# Autodesk Inventor assembly: Additional_Building
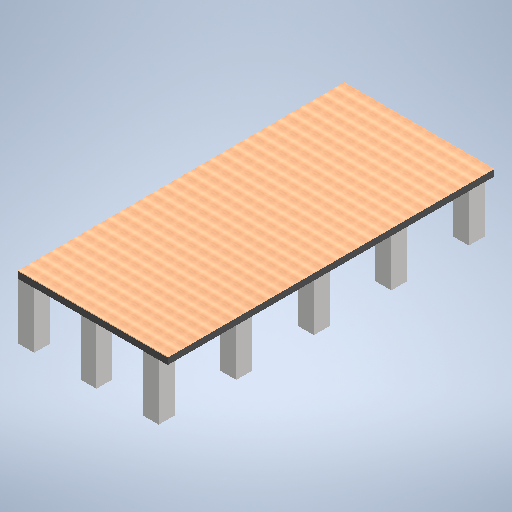
[picture p0: Inventor's stored thumbnail of the model, 512x512]
Saved by Autodesk Inventor 2025 (Build 290162010, 162A)
## iProperties
Created: 2024-08-02
Part Number: Additional_Building
Document SubType Name: Assembly
Designer: Tom
Author: Tom
## Documents named in this file (3)
- C:\Users\Tom\Documents\Inventor\Mobility\Additional_Building\Additional_Building.iam
- C:\Users\Tom\Documents\Inventor\Mobility\Additional_Building\Grid_Of_Piers.iam
- C:\Users\Tom\Documents\Inventor\Mobility\Additional_Building\Floor_System.iam
## Components (2 placed, 2 different names)
1. Grid_Of_Piers:1 [sub-assembly] — Mate:12, Mate:13, Flush:7
2. Floor_System:1 [sub-assembly] — Mate:12, Mate:13, Flush:7
## Relationships (3: Mate 2, Flush 1)
- Mate:12: Grid_Of_Piers:1 ↔ Floor_System:1
- Mate:13: Grid_Of_Piers:1 ↔ Floor_System:1
- Flush:7: Grid_Of_Piers:1 ↔ Floor_System:1
